# Autodesk Inventor assembly: gripper_hand_connector
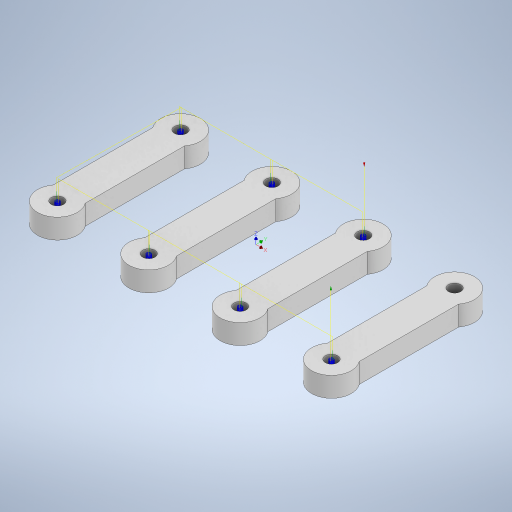
[picture p0: Inventor's stored thumbnail of the model, 512x512]
Saved by Autodesk Inventor 2024.2 (Build 282272000, 272)
## iProperties
Created: 2024-01-08
Part Number: gripper_hand_connector
Document SubType Name: Assembly
Designer: chanh
Author: chanh
## Documents named in this file (2)
- C:\Users\chanh\내 드라이브\로봇\Humanoid\Roboin Humanoid Project\Inventor\rh_plus_7_axis_robot_arm_hardware\CAM\5T\gripper_hand_connector.iam
- C:\Users\chanh\내 드라이브\로봇\Humanoid\Roboin Humanoid Project\Inventor\rh_plus_7_axis_robot_arm_hardware\CAM\5T\gripper_hand_connector.ipt
## Components (4 placed, 1 different names)
1. gripper_hand_connector:1 — Mate:1, Mate:2, Flush:1, Mate:3, Flush:2, Flush:3, Flush:4, Flush:5, Flush:6, Flush:7
2. gripper_hand_connector:2 — Mate:3, Mate:4, Flush:2, Flush:5
3. gripper_hand_connector:3 — Mate:4, Mate:5, Flush:3, Flush:6
4. gripper_hand_connector:4 — Mate:5, Flush:4, Flush:7
## Relationships (12: Flush 7, Mate 5)
- Mate:1: gripper_hand_connector:1
- Mate:2: gripper_hand_connector:1
- Flush:1: gripper_hand_connector:1
- Mate:3 (15 mm): gripper_hand_connector:1 ↔ gripper_hand_connector:2
- Mate:4 (15 mm): gripper_hand_connector:2 ↔ gripper_hand_connector:3
- Mate:5 (15 mm): gripper_hand_connector:3 ↔ gripper_hand_connector:4
- Flush:2: gripper_hand_connector:1 ↔ gripper_hand_connector:2
- Flush:3: gripper_hand_connector:1 ↔ gripper_hand_connector:3
- Flush:4: gripper_hand_connector:1 ↔ gripper_hand_connector:4
- Flush:5: gripper_hand_connector:1 ↔ gripper_hand_connector:2
- Flush:6: gripper_hand_connector:1 ↔ gripper_hand_connector:3
- Flush:7: gripper_hand_connector:1 ↔ gripper_hand_connector:4
